# Autodesk Inventor assembly: XRevit Filter column D940
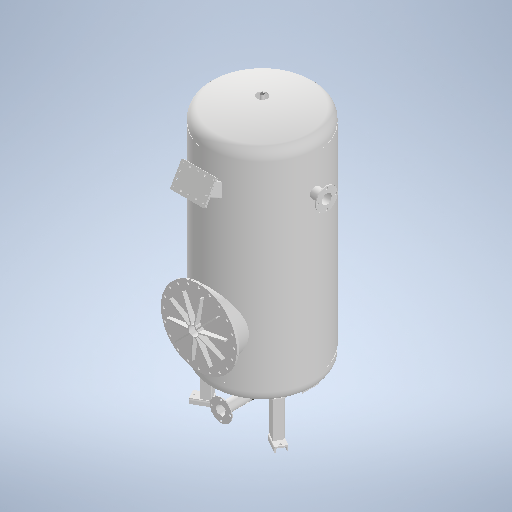
[picture p0: Inventor's stored thumbnail of the model, 512x512]
Saved by Autodesk Inventor 2025 (Build 290162010, 162A)
## iProperties
allow_slope_adjustment: 0 ul
flow_configuration2: 1 ul
flow_direction: 2 ul
loss_method: 0 ul
radius: 45,500 mm
Created: 2025-02-13
Part Number: XRevit Filter column D940
Document SubType Name: Assembly
Designer: pokla
Mass: 370112 g
Surface Area: 188070 cm^2
Volume: 53414.8 cm^3
Density: 6.92901 g/cm^3
radius: 16,750 mm
Author: pokla
Revision Number: 3
## Documents named in this file (23)
- C:\Users\pokla\Documents\Inventor\PRS-Purovskii\Model\PRS-filter 940\ASY PRS Filter column D940.iam
- C:\Users\pokla\Documents\Inventor\PRS-Purovskii\Model\PRS-filter 940\PRS 940-22 accses hatch flangeipt.ipt
- C:\Users\pokla\Documents\Inventor\PRS-Purovskii\Model\PRS-filter 940\PRS 940-11 accses hatch tube.ipt
- C:\Users\pokla\Documents\Inventor\PRS-Purovskii\Model\PRS-filter 940\PRS 940-02 dished head.ipt
- C:\Users\pokla\Documents\Inventor\PRS-Purovskii\Model\PRS-filter 940\Fitting G1.ipt
- C:\Users\pokla\Documents\Inventor\PRS-Purovskii\Model\PRS-filter 940\ASY PRS 940-90 Filter legs.iam
- C:\Users\pokla\Documents\Inventor\PRS-Purovskii\Model\PRS-filter 940\PRS 940-33 charging blind flange.ipt
- C:\Users\pokla\Documents\Inventor\PRS-Purovskii\Model\PRS-filter 940\ASY PRS 940-20 charging hatch.iam
- C:\Users\pokla\Documents\Inventor\PRS-Purovskii\Model\PRS-filter 940\PRS 940-12 FDS tube 2.ipt
- C:\Users\pokla\Documents\Inventor\PRS-Purovskii\Model\PRS-filter 940\PRS 940-06 charging flange round.ipt
- C:\Users\pokla\Documents\Inventor\PRS-Purovskii\Model\PRS-filter 940\PRS 940-13 FDS tube 3.ipt
- C:\Users\pokla\Documents\Inventor\PRS-Purovskii\Model\PRS-filter 940\PRS 940-14 FDS tube 4.ipt
- C:\Users\pokla\Documents\Inventor\PRS-Purovskii\Model\PRS-filter 940\PRS 940-15 FDS tube 5.ipt
- C:\Users\pokla\Documents\Inventor\PRS-Purovskii\Model\PRS-filter 940\PRS 940-31 FDS flange DN90.ipt
- C:\Users\pokla\Documents\Inventor\PRS-Purovskii\Model\PRS-filter 940\PRS 940-32 FDS free flange DN90.ipt
- C:\Users\pokla\Documents\Inventor\PRS-Purovskii\Model\PRS-filter 940\PRS 940-71 charging tube 1.ipt
- C:\Users\pokla\Documents\Inventor\PRS-Purovskii\Model\PRS-filter 940\PRS 940-72 charging tube 2.ipt
- C:\Users\pokla\Documents\Inventor\PRS-Purovskii\Model\PRS-filter 940\PRS 940-07 charging flange rect.ipt
- C:\Users\pokla\Documents\Inventor\PRS-Purovskii\Model\PRS-filter 940\PRS 940-10 main Shell D 940.ipt
- C:\Users\pokla\Documents\Inventor\PRS-Purovskii\Model\PRS-filter 940\JIS B 2312 90 Deg Long Elbow Steel 50A x Sch 40.ipt
- C:\Users\pokla\Documents\Inventor\PRS-Purovskii\Model\PRS-filter 940\ASY PRS 940-80 top funnel.iam
- C:\Users\pokla\Documents\Inventor\PRS-Purovskii\Model\PRS-filter 940\ASY PRS 940-50 filter-distribution-system.iam
- C:\Users\pokla\Documents\Inventor\Content Center Files\R2025\en-US\JIS B 2312 90 (2)\JIS B 2312 90 Deg Long Elbow Steel 80A x Sch 40.ipt
## Components (28 placed, 22 different names)
1. Fitting G1.ipt:1 — Rigid:15
2. PRS 940-33 charging blind flange.ipt:1 — Rigid:67
3. PRS 940-10 main Shell D 940.ipt:1 — Flush:7, Rigid:85, Flush:8, Rotational:76, Rotational:77, Rigid:86, Rigid:87
4. PRS 940-33 charging blind flange.ipt:2 — Rigid:77
5. PRS 940-33 charging blind flange.ipt:3 — Rigid:78, Rigid:90
6. PRS 940-02 dished head.ipt:2 — Rotational:77, Rigid:88, Mate:7
7. Fitting G1.ipt:2 — Mate:4, Mate:5, Mate:6
8. JIS B 2312 90 Deg Long Elbow Steel 80A x Sch 40.ipt:1 — Rigid:68, Rigid:79, Mate:6, Rigid:88
9. PRS 940-13 FDS tube 3.ipt:1 — Rigid:67, Rigid:68, Flush:9
10. PRS 940-14 FDS tube 4.ipt:1 — Rigid:79, Rotational:71
11. PRS 940-31 FDS flange DN90.ipt:1 — Rigid:76
12. PRS 940-32 FDS free flange DN90.ipt:1 — Rotational:71, Rigid:76, Rotational:78
13. PRS 940-11 accses hatch tube.ipt:1 — Rotational:74, Rigid:85
14. PRS 940-02 dished head.ipt:1 — Rigid:15, Rotational:76
15. JIS B 2312 90 Deg Long Elbow Steel 50A x Sch 40.ipt:1 — Rigid:62, Rigid:73
16. PRS 940-12 FDS tube 2.ipt:1 — Rigid:62, Rigid:78
17. PRS 940-15 FDS tube 5.ipt:1 — Rigid:73, Rigid:77, Rigid:87
18. PRS 940-72 charging tube 2.ipt:1 — Rigid:84, Rigid:89
19. PRS 940-71 charging tube 1.ipt:1 — Rigid:84, Rigid:86
20. PRS 940-06 charging flange round.ipt:1 — Rigid:83, Rigid:89
21. PRS 940-07 charging flange rect.ipt:1 — Rigid:83
22. PRS 940-22 accses hatch flangeipt.ipt:1 — Rotational:73, Rotational:74
23. ASY PRS 940-20 charging hatch.iam:1 [sub-assembly] — Rotational:73
24. ASY PRS 940-80 top funnel.iam:1 [sub-assembly] — Rigid:90
25. ASY PRS 940-50 filter-distribution-system.iam:1 [sub-assembly] — Rotational:78
26. ASY PRS 940-90 Filter legs.iam:1 [sub-assembly] — Flush:2, Flush:10, Flush:11
27. ASY PRS 940-90 Filter legs.iam:2 [sub-assembly]
28. ASY PRS 940-90 Filter legs.iam:3 [sub-assembly]
## Component patterns: (3 elements, first: ASY PRS 940-90 Filter legs.iam:1)
## Relationships (33: WeldJoint 17, Flush 6, RevoluteJoint 6, Mate 4)
- Rigid:15 [WeldJoint]: Fitting G1.ipt:1 ↔ PRS 940-02 dished head.ipt:1
- Flush:2: ASY PRS 940-90 Filter legs.iam:1
- Rigid:62 [WeldJoint]: JIS B 2312 90 Deg Long Elbow Steel 50A x Sch 40.ipt:1 ↔ PRS 940-12 FDS tube 2.ipt:1
- Rigid:67 [WeldJoint]: PRS 940-33 charging blind flange.ipt:1 ↔ PRS 940-13 FDS tube 3.ipt:1
- Rigid:68 [WeldJoint]: JIS B 2312 90 Deg Long Elbow Steel 80A x Sch 40.ipt:1 ↔ PRS 940-13 FDS tube 3.ipt:1
- Rigid:79 [WeldJoint] (1 mm): JIS B 2312 90 Deg Long Elbow Steel 80A x Sch 40.ipt:1 ↔ PRS 940-14 FDS tube 4.ipt:1
- Rigid:73 [WeldJoint]: JIS B 2312 90 Deg Long Elbow Steel 50A x Sch 40.ipt:1 ↔ PRS 940-15 FDS tube 5.ipt:1
- Rotational:71 [RevoluteJoint]: PRS 940-14 FDS tube 4.ipt:1 ↔ PRS 940-32 FDS free flange DN90.ipt:1
- Rigid:76 [WeldJoint]: PRS 940-31 FDS flange DN90.ipt:1 ↔ PRS 940-32 FDS free flange DN90.ipt:1
- Rigid:77 [WeldJoint]: PRS 940-33 charging blind flange.ipt:2 ↔ PRS 940-15 FDS tube 5.ipt:1
- Rigid:78 [WeldJoint]: PRS 940-33 charging blind flange.ipt:3 ↔ PRS 940-12 FDS tube 2.ipt:1
- Rotational:73 [RevoluteJoint]: PRS 940-22 accses hatch flangeipt.ipt:1 ↔ ASY PRS 940-20 charging hatch.iam:1
- Rotational:74 [RevoluteJoint]: PRS 940-11 accses hatch tube.ipt:1 ↔ PRS 940-22 accses hatch flangeipt.ipt:1
- Rigid:83 [WeldJoint]: PRS 940-06 charging flange round.ipt:1 ↔ PRS 940-07 charging flange rect.ipt:1
- Rigid:84 [WeldJoint]: PRS 940-72 charging tube 2.ipt:1 ↔ PRS 940-71 charging tube 1.ipt:1
- Flush:10: ASY PRS 940-90 Filter legs.iam:1
- Flush:11: ASY PRS 940-90 Filter legs.iam:1
- Flush:7: PRS 940-10 main Shell D 940.ipt:1
- Rigid:85 [WeldJoint]: PRS 940-10 main Shell D 940.ipt:1 ↔ PRS 940-11 accses hatch tube.ipt:1
- Flush:8: PRS 940-10 main Shell D 940.ipt:1
- Rotational:76 [RevoluteJoint]: PRS 940-10 main Shell D 940.ipt:1 ↔ PRS 940-02 dished head.ipt:1
- Rotational:77 [RevoluteJoint]: PRS 940-10 main Shell D 940.ipt:1 ↔ PRS 940-02 dished head.ipt:2
- Flush:9: PRS 940-13 FDS tube 3.ipt:1
- Rigid:86 [WeldJoint]: PRS 940-10 main Shell D 940.ipt:1 ↔ PRS 940-71 charging tube 1.ipt:1
- Rigid:87 [WeldJoint] (100 mm): PRS 940-10 main Shell D 940.ipt:1 ↔ PRS 940-15 FDS tube 5.ipt:1
- Mate:4: Fitting G1.ipt:2
- Mate:5 (150 mm): Fitting G1.ipt:2
- Mate:6: Fitting G1.ipt:2 ↔ JIS B 2312 90 Deg Long Elbow Steel 80A x Sch 40.ipt:1
- Rigid:88 [WeldJoint] (1 mm): PRS 940-02 dished head.ipt:2 ↔ JIS B 2312 90 Deg Long Elbow Steel 80A x Sch 40.ipt:1
- Rigid:89 [WeldJoint]: PRS 940-72 charging tube 2.ipt:1 ↔ PRS 940-06 charging flange round.ipt:1
- Rigid:90 [WeldJoint]: PRS 940-33 charging blind flange.ipt:3 ↔ ASY PRS 940-80 top funnel.iam:1
- Rotational:78 [RevoluteJoint]: PRS 940-32 FDS free flange DN90.ipt:1 ↔ ASY PRS 940-50 filter-distribution-system.iam:1
- Mate:7 (300 mm): PRS 940-02 dished head.ipt:2
